# Autodesk Inventor assembly: Test tube
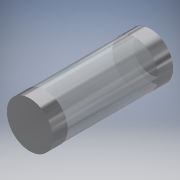
[picture p0: Inventor's stored thumbnail of the model, 180x180]
Saved by Autodesk Inventor 2017 (Build 210142000, 142)
## iProperties
Created: 2017-06-10
Part Number: Test tube
Document SubType Name: Assembly
Designer: Blaire Weinberg
Author: Blaire Weinberg
## Documents named in this file (4)
- C:\UMD\BPP\ROCKSAT X\star\CAD\Mechanical\Full payload assembly\Subsystems\Test Tube Rack\Test tube.iam
- C:\UMD\BPP\ROCKSAT X\star\CAD\Mechanical\Full payload assembly\Subsystems\Test Tube Rack\Test Tube.ipt
- C:\UMD\BPP\ROCKSAT X\star\CAD\Mechanical\Full payload assembly\Subsystems\Test Tube Rack\Wire Mesh.ipt
- C:\UMD\BPP\ROCKSAT X\star\CAD\Mechanical\Full payload assembly\Subsystems\Test Tube Rack\Aluminum Foil.ipt
## Components (5 placed, 3 different names)
1. Test Tube:1 — Mate:1, Mate:2, Mate:3, Mate:4, Mate:6, Mate:8
2. Wire Mesh:1 — Mate:1, Mate:2, Mate:7
3. Wire Mesh:2 — Mate:3, Mate:4, Mate:5
4. Aluminum Foil:1 — Mate:5, Mate:6
5. Aluminum Foil:2 — Mate:7, Mate:8
## Relationships (8: Mate 8)
- Mate:1: Test Tube:1 ↔ Wire Mesh:1
- Mate:2: Test Tube:1 ↔ Wire Mesh:1
- Mate:3: Test Tube:1 ↔ Wire Mesh:2
- Mate:4: Test Tube:1 ↔ Wire Mesh:2
- Mate:5: Wire Mesh:2 ↔ Aluminum Foil:1
- Mate:6: Test Tube:1 ↔ Aluminum Foil:1
- Mate:7: Wire Mesh:1 ↔ Aluminum Foil:2
- Mate:8: Test Tube:1 ↔ Aluminum Foil:2
